# Autodesk Inventor assembly: hand5
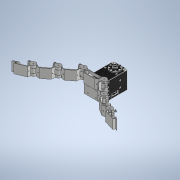
[picture p0: Inventor's stored thumbnail of the model, 180x180]
Saved by Autodesk Inventor 2021 (Build 250183000, 183)
## iProperties
Created: 2022-09-22
Part Number: hand5
Document SubType Name: Assembly
Designer: ereg140
Author: ereg140
## Documents named in this file (6)
- \\files.auckland.ac.nz\myhome\Documents\GitHub\hand\PRINTS\hand5.iam
- \\files.auckland.ac.nz\myhome\Documents\GitHub\hand\Phalalnge5_palm_dynamixel.ipt
- \\files.auckland.ac.nz\myhome\Documents\GitHub\hand\XM430 Motor\XM430-Working-Shaft.iam
- \\files.auckland.ac.nz\myhome\Documents\GitHub\hand\Palm Spacer.ipt
- \\files.auckland.ac.nz\myhome\Documents\GitHub\hand\Phalalnge5_35mm.ipt
- \\files.auckland.ac.nz\myhome\Documents\GitHub\hand\Phalalnge5_35mm_TIP.ipt
## Components (9 placed, 5 different names)
1. Phalalnge5_palm_dynamixel:1 — Rigid:4, Flush:2, Cylindrical:2, Flush:6, Cylindrical:6
2. XM430-Working-Shaft:1 [sub-assembly] — Rigid:3
3. Palm Spacer:1 — Rigid:3, Rigid:4
4. Phalalnge5_35mm:1 — Flush:1, Cylindrical:1, Flush:3, Cylindrical:3
5. Phalalnge5_35mm:2 — Flush:1, Cylindrical:1, Flush:2, Cylindrical:2
6. Phalalnge5_35mm_TIP:1 — Flush:3, Cylindrical:3
7. Phalalnge5_35mm:3
8. Phalalnge5_35mm:4 — Flush:6, Cylindrical:6
9. Phalalnge5_35mm_TIP:2
## Relationships (14: Flush 6, CylindricalJoint 6, WeldJoint 2)
- Rigid:3 [WeldJoint]: XM430-Working-Shaft:1 ↔ Palm Spacer:1
- Rigid:4 [WeldJoint]: Phalalnge5_palm_dynamixel:1 ↔ Palm Spacer:1
- Flush:1: Phalalnge5_35mm:1 ↔ Phalalnge5_35mm:2
- Cylindrical:1: Phalalnge5_35mm:1 ↔ Phalalnge5_35mm:2
- Flush:2: Phalalnge5_palm_dynamixel:1 ↔ Phalalnge5_35mm:2
- Cylindrical:2: Phalalnge5_palm_dynamixel:1 ↔ Phalalnge5_35mm:2
- Flush:3: Phalalnge5_35mm:1 ↔ Phalalnge5_35mm_TIP:1
- Cylindrical:3: Phalalnge5_35mm:1 ↔ Phalalnge5_35mm_TIP:1
- [Flush]: Phalalnge5_35mm:3 ↔ Phalalnge5_35mm:4
- [CylindricalJoint]: Phalalnge5_35mm:3 ↔ Phalalnge5_35mm:4
- [Flush]: Phalalnge5_35mm:3 ↔ Phalalnge5_35mm_TIP:2
- [CylindricalJoint]: Phalalnge5_35mm:3 ↔ Phalalnge5_35mm_TIP:2
- Flush:6: Phalalnge5_palm_dynamixel:1 ↔ Phalalnge5_35mm:4
- Cylindrical:6: Phalalnge5_palm_dynamixel:1 ↔ Phalalnge5_35mm:4
## Named parameters: d16_d15 = 4.7 mm, d17_d7 = 0 mm, d18_d8 = 44.048008 deg, d19_d9 = -4.7 mm, d20_d13 = 0 mm, d21_d14 = 131.939982 deg
